# Autodesk Inventor assembly: termoformadora
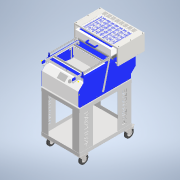
[picture p0: Inventor's stored thumbnail of the model, 180x180]
Saved by Autodesk Inventor 2021 (Build 250183000, 183)
## iProperties
Created: 2021-04-15
Part Number: termoformadora
Document SubType Name: Assembly
Designer: Leonardo Fabio Mercado Benítez
Author: Leonardo Fabio Mercado Benítez
## Documents named in this file (21)
- C:\Users\Nelson\Github\Proyecto_PAI_2021\01 CAD\termoformadora.iam
- C:\Users\Nelson\Github\Proyecto_PAI_2021\01 CAD\soporte_inferior_zona_calor.ipt
- C:\Users\Nelson\Github\Proyecto_PAI_2021\01 CAD\tapa_caja_calor.ipt
- C:\Users\Nelson\Github\Proyecto_PAI_2021\01 CAD\angulo_caja_calor.ipt
- C:\Users\Nelson\Github\Proyecto_PAI_2021\01 CAD\buje_carro_zona_calor.ipt
- C:\Users\Nelson\Github\Proyecto_PAI_2021\01 CAD\barra.ipt
- C:\Users\Nelson\Github\Proyecto_PAI_2021\01 CAD\mango_zona_calor.ipt
- C:\Users\Nelson\Github\Proyecto_PAI_2021\01 CAD\Ensamblaje carcasa control.iam
- C:\Users\Nelson\Github\Proyecto_PAI_2021\01 CAD\soporte_barra.ipt
- C:\Users\Nelson\Github\Proyecto_PAI_2021\01 CAD\ensamble resistencias.iam
- C:\Users\Nelson\Github\Proyecto_PAI_2021\01 CAD\soporte_resistencias.ipt
- C:\Users\Nelson\Github\Proyecto_PAI_2021\01 CAD\Estructura Lámina.iam
- C:\Users\Nelson\Github\Proyecto_PAI_2021\01 CAD\conector_ceramico.ipt
- C:\Users\Nelson\Github\Proyecto_PAI_2021\01 CAD\guarda_conector_ceramico.ipt
- C:\Users\Nelson\Github\Proyecto_PAI_2021\01 CAD\guarda_cables.ipt
- C:\Users\Nelson\Github\Proyecto_PAI_2021\01 CAD\Barras_Soporte_superior.ipt
- C:\Users\Admin\Documents\Inventor\Content Center Files\R2021\es-ES\ISO 7380-1\ISO 7380-1 - M5 x 16.ipt
- C:\Users\Nelson\Github\Proyecto_PAI_2021\01 CAD\DIN EN ISO 7049 - ST2,9 x 6,5 - C - H.ipt
- C:\Users\Nelson\Github\Proyecto_PAI_2021\01 CAD\Tuerca-1_4.ipt
- C:\Users\Nelson\Github\Proyecto_PAI_2021\01 CAD\Tornillo1_4x1_2.ipt
- C:\Users\Nelson\Github\Proyecto_PAI_2021\01 CAD\Ensamblaje_Carcaza_sup_ch.iam
## Components (55 placed, 20 different names)
1. soporte_inferior_zona_calor:1 — Coincidencia:3, Coincidencia:5, Nivelación:3, Nivelación:4, Coincidencia:6, Nivelación:5, Nivelación:6, Coincidencia:15, Insertar:5, Insertar:6, Coincidencia:44, Coincidencia:45, Nivelación:14, Nivelación:15, Ángulo:6, Ángulo:7, Ángulo:8, Ángulo:9, Ángulo:10, Nivelación:16, Coincidencia:56, Nivelación:17
2. tapa_caja_calor:1 — Coincidencia:3, Nivelación:14, Nivelación:15, De rotación:1, De rotación:2, De rotación:3, De rotación:4
3. angulo_caja_calor:1 — Coincidencia:5, Nivelación:3, Nivelación:4, Coincidencia:7, Coincidencia:8, Insertar:1, Insertar:2
4. angulo_caja_calor:2 — Coincidencia:6, Nivelación:5, Nivelación:6, Coincidencia:9, Coincidencia:10, Insertar:3, Insertar:4
5. buje_carro_zona_calor:1 — Coincidencia:9, Insertar:3
6. buje_carro_zona_calor:2 — Coincidencia:8, Insertar:2, Coincidencia:14
7. buje_carro_zona_calor:3 — Coincidencia:10, Insertar:4
8. buje_carro_zona_calor:4 — Coincidencia:7, Insertar:1, Coincidencia:13
9. barra:1 — Coincidencia:13, Coincidencia:21
10. barra:2 — Coincidencia:14, Coincidencia:22
11. mango_zona_calor:1 — Coincidencia:15, Insertar:5, Insertar:6
12. Ensamblaje carcasa control:1 [sub-assembly] — Nivelación:8, Coincidencia:18, Coincidencia:20, Nivelación:9, Coincidencia:23, Coincidencia:33, Nivelación:10, Nivelación:11, Rígido:1, Rígido:2, Rígido:3, Rígido:4
13. soporte_barra:1 — Nivelación:8, Coincidencia:18, Coincidencia:22
14. soporte_barra:2 — Coincidencia:20, Nivelación:9, Coincidencia:21
15. ensamble resistencias:1 [sub-assembly] — Coincidencia:23, Coincidencia:29, Nivelación:12, Nivelación:13, Coincidencia:73, Coincidencia:74, Coincidencia:75, Coincidencia:76, Coincidencia:77, Coincidencia:78, Coincidencia:79, Coincidencia:80, Coincidencia:81, Coincidencia:82, Coincidencia:83, Coincidencia:84
16. soporte_resistencias:1 — Coincidencia:29, Nivelación:12, Nivelación:13, Coincidencia:34, Coincidencia:35, Coincidencia:36, Coincidencia:37, Coincidencia:38, Coincidencia:39, Coincidencia:40, Coincidencia:41, Coincidencia:42, Coincidencia:43, Ángulo:1, Ángulo:2, Ángulo:3, Ángulo:4, Ángulo:5, Coincidencia:44, Coincidencia:45, Coincidencia:61, Coincidencia:62, Coincidencia:63, Coincidencia:64, Coincidencia:65, Coincidencia:66, Coincidencia:67, Coincidencia:68, Coincidencia:69, Coincidencia:70, Coincidencia:71, Coincidencia:72
17. Estructura Lámina:1 [sub-assembly] — Coincidencia:33, Nivelación:10, Nivelación:11
18. conector_ceramico:1 — Coincidencia:37, Coincidencia:42, Ángulo:2, Coincidencia:52, Coincidencia:91
19. conector_ceramico:2 — Coincidencia:36, Coincidencia:41, Ángulo:1, Coincidencia:53, Coincidencia:94
20. conector_ceramico:3 — Coincidencia:34, Coincidencia:39, Ángulo:4, Coincidencia:55, Coincidencia:92
21. conector_ceramico:4 — Coincidencia:38, Coincidencia:43, Ángulo:5, Coincidencia:46, Coincidencia:47, Coincidencia:48, Coincidencia:49, Coincidencia:50, Coincidencia:51, Coincidencia:90
22. conector_ceramico:5 — Coincidencia:35, Coincidencia:40, Ángulo:3, Coincidencia:54, Coincidencia:93
23. guarda_conector_ceramico:1 — Coincidencia:46, Coincidencia:51, Ángulo:10, Coincidencia:89
24. guarda_conector_ceramico:2 — Coincidencia:48, Coincidencia:54, Ángulo:8, Coincidencia:86
25. guarda_conector_ceramico:3 — Coincidencia:47, Coincidencia:52, Ángulo:6, Coincidencia:88
26. guarda_conector_ceramico:4 — Coincidencia:50, Coincidencia:55, Ángulo:9, Coincidencia:87
27. guarda_conector_ceramico:5 — Coincidencia:49, Coincidencia:53, Ángulo:7, Coincidencia:85
28. guarda_cables:1 — Nivelación:16, Coincidencia:56, Nivelación:17
29. Barras_Soporte_superior:1 — Rígido:4
30. Barras_Soporte_superior:2 — Rígido:3
31. Barras_Soporte_superior:3 — Rígido:1
32. Barras_Soporte_superior:4 — Rígido:2, Coincidencia:95
33. ISO 7380-1 M5 x 16:4
34. DIN EN ISO 7049 - C-H ST2,9 x 6,5 - C - H:1 — De rotación:2
35. DIN EN ISO 7049 - C-H ST2,9 x 6,5 - C - H:2 — De rotación:1
36. DIN EN ISO 7049 - C-H ST2,9 x 6,5 - C - H:3 — De rotación:4
37. DIN EN ISO 7049 - C-H ST2,9 x 6,5 - C - H:4 — De rotación:3
38. AS 2465 - Pulgadas 1/4  UNC:1 — Coincidencia:61, Coincidencia:74
39. AS 2465 - Pulgadas 1/4  UNC:2 — Coincidencia:62, Coincidencia:76
40. AS 2465 - Pulgadas 1/4  UNC:3 — Coincidencia:64, Coincidencia:79
41. AS 2465 - Pulgadas 1/4  UNC:4 — Coincidencia:63, Coincidencia:75
42. AS 2465 - Pulgadas 1/4  UNC:5 — Coincidencia:65, Coincidencia:77
43. AS 2465 - Pulgadas 1/4  UNC:6 — Coincidencia:68, Coincidencia:80
44. AS 2465 - Pulgadas 1/4  UNC:7 — Coincidencia:69, Coincidencia:81
45. AS 2465 - Pulgadas 1/4  UNC:8 — Coincidencia:67, Coincidencia:78
46. AS 2465 - Pulgadas 1/4  UNC:9 — Coincidencia:66, Coincidencia:73
47. AS 2465 - Pulgadas 1/4  UNC:10 — Coincidencia:70, Coincidencia:82
48. AS 2465 - Pulgadas 1/4  UNC:11 — Coincidencia:72, Coincidencia:84
49. AS 2465 - Pulgadas 1/4  UNC:12 — Coincidencia:71, Coincidencia:83
50. AS 2465 - Pulgadas 1/4 x 1/2  UNC:1 — Coincidencia:85, Coincidencia:94
51. AS 2465 - Pulgadas 1/4 x 1/2  UNC:2 — Coincidencia:88, Coincidencia:93
52. AS 2465 - Pulgadas 1/4 x 1/2  UNC:3 — Coincidencia:87, Coincidencia:91
53. AS 2465 - Pulgadas 1/4 x 1/2  UNC:4 — Coincidencia:89, Coincidencia:90
54. AS 2465 - Pulgadas 1/4 x 1/2  UNC:5 — Coincidencia:86, Coincidencia:92
55. Ensamblaje_Carcaza_sup_ch:1 [sub-assembly] — Coincidencia:95
## Relationships (113: Mate 75, Flush 14, Angle 10, Insert 6, RevoluteJoint 4, WeldJoint 4)
- Coincidencia:3 [Mate]: soporte_inferior_zona_calor:1 ↔ tapa_caja_calor:1
- Coincidencia:5 [Mate]: soporte_inferior_zona_calor:1 ↔ angulo_caja_calor:1
- Nivelación:3 [Flush]: soporte_inferior_zona_calor:1 ↔ angulo_caja_calor:1
- Nivelación:4 [Flush] (10 mm): soporte_inferior_zona_calor:1 ↔ angulo_caja_calor:1
- Coincidencia:6 [Mate]: soporte_inferior_zona_calor:1 ↔ angulo_caja_calor:2
- Nivelación:5 [Flush]: soporte_inferior_zona_calor:1 ↔ angulo_caja_calor:2
- Nivelación:6 [Flush]: soporte_inferior_zona_calor:1 ↔ angulo_caja_calor:2
- Coincidencia:7 [Mate]: angulo_caja_calor:1 ↔ buje_carro_zona_calor:4
- Coincidencia:8 [Mate]: angulo_caja_calor:1 ↔ buje_carro_zona_calor:2
- Coincidencia:9 [Mate]: angulo_caja_calor:2 ↔ buje_carro_zona_calor:1
- Coincidencia:10 [Mate]: angulo_caja_calor:2 ↔ buje_carro_zona_calor:3
- Insertar:1: angulo_caja_calor:1 ↔ buje_carro_zona_calor:4
- Insertar:2: angulo_caja_calor:1 ↔ buje_carro_zona_calor:2
- Insertar:3: angulo_caja_calor:2 ↔ buje_carro_zona_calor:1
- Insertar:4: angulo_caja_calor:2 ↔ buje_carro_zona_calor:3
- Coincidencia:13 [Mate]: buje_carro_zona_calor:4 ↔ barra:1
- Coincidencia:14 [Mate]: buje_carro_zona_calor:2 ↔ barra:2
- Coincidencia:15 [Mate]: soporte_inferior_zona_calor:1 ↔ mango_zona_calor:1
- Insertar:5: soporte_inferior_zona_calor:1 ↔ mango_zona_calor:1
- Insertar:6: soporte_inferior_zona_calor:1 ↔ mango_zona_calor:1
- Nivelación:8 [Flush] (5 mm): Ensamblaje carcasa control:1 ↔ soporte_barra:1
- Coincidencia:18 [Mate]: Ensamblaje carcasa control:1 ↔ soporte_barra:1
- Coincidencia:20 [Mate]: Ensamblaje carcasa control:1 ↔ soporte_barra:2
- Nivelación:9 [Flush] (5 mm): Ensamblaje carcasa control:1 ↔ soporte_barra:2
- Coincidencia:21 [Mate]: barra:1 ↔ soporte_barra:2
- Coincidencia:22 [Mate]: barra:2 ↔ soporte_barra:1
- Coincidencia:23 [Mate] (106 mm): Ensamblaje carcasa control:1 ↔ ensamble resistencias:1
- Coincidencia:29 [Mate]: ensamble resistencias:1 ↔ soporte_resistencias:1
- Coincidencia:33 [Mate]: Ensamblaje carcasa control:1 ↔ Estructura Lámina:1
- Nivelación:10 [Flush] (10 mm): Ensamblaje carcasa control:1 ↔ Estructura Lámina:1
- Nivelación:11 [Flush]: Ensamblaje carcasa control:1 ↔ Estructura Lámina:1
- Nivelación:12 [Flush] (33.5 mm): ensamble resistencias:1 ↔ soporte_resistencias:1
- Nivelación:13 [Flush] (34 mm): ensamble resistencias:1 ↔ soporte_resistencias:1
- Coincidencia:34 [Mate]: soporte_resistencias:1 ↔ conector_ceramico:3
- Coincidencia:35 [Mate]: soporte_resistencias:1 ↔ conector_ceramico:5
- Coincidencia:36 [Mate]: soporte_resistencias:1 ↔ conector_ceramico:2
- Coincidencia:37 [Mate]: soporte_resistencias:1 ↔ conector_ceramico:1
- Coincidencia:38 [Mate]: soporte_resistencias:1 ↔ conector_ceramico:4
- Coincidencia:39 [Mate]: soporte_resistencias:1 ↔ conector_ceramico:3
- Coincidencia:40 [Mate]: soporte_resistencias:1 ↔ conector_ceramico:5
- Coincidencia:41 [Mate]: soporte_resistencias:1 ↔ conector_ceramico:2
- Coincidencia:42 [Mate]: soporte_resistencias:1 ↔ conector_ceramico:1
- Coincidencia:43 [Mate]: soporte_resistencias:1 ↔ conector_ceramico:4
- Ángulo:1 [Angle] (0 deg): soporte_resistencias:1 ↔ conector_ceramico:2
- Ángulo:2 [Angle] (0 deg): soporte_resistencias:1 ↔ conector_ceramico:1
- Ángulo:3 [Angle] (0 deg): soporte_resistencias:1 ↔ conector_ceramico:5
- Ángulo:4 [Angle] (0 deg): soporte_resistencias:1 ↔ conector_ceramico:3
- Ángulo:5 [Angle] (0 deg): soporte_resistencias:1 ↔ conector_ceramico:4
- Coincidencia:44 [Mate] (0.5 mm): soporte_inferior_zona_calor:1 ↔ soporte_resistencias:1
- Coincidencia:45 [Mate] (0.5 mm): soporte_inferior_zona_calor:1 ↔ soporte_resistencias:1
- Nivelación:14 [Flush] (25.4 mm): soporte_inferior_zona_calor:1 ↔ tapa_caja_calor:1
- Nivelación:15 [Flush] (31.75 mm): soporte_inferior_zona_calor:1 ↔ tapa_caja_calor:1
- Coincidencia:46 [Mate]: conector_ceramico:4 ↔ guarda_conector_ceramico:1
- Coincidencia:47 [Mate]: conector_ceramico:4 ↔ guarda_conector_ceramico:3
- Coincidencia:48 [Mate]: conector_ceramico:4 ↔ guarda_conector_ceramico:2
- Coincidencia:49 [Mate]: conector_ceramico:4 ↔ guarda_conector_ceramico:5
- Coincidencia:50 [Mate]: conector_ceramico:4 ↔ guarda_conector_ceramico:4
- Coincidencia:51 [Mate]: conector_ceramico:4 ↔ guarda_conector_ceramico:1
- Coincidencia:52 [Mate]: conector_ceramico:1 ↔ guarda_conector_ceramico:3
- Coincidencia:53 [Mate]: conector_ceramico:2 ↔ guarda_conector_ceramico:5
- Coincidencia:54 [Mate]: conector_ceramico:5 ↔ guarda_conector_ceramico:2
- Coincidencia:55 [Mate]: conector_ceramico:3 ↔ guarda_conector_ceramico:4
- Ángulo:6 [Angle] (0 deg): soporte_inferior_zona_calor:1 ↔ guarda_conector_ceramico:3
- Ángulo:7 [Angle] (0 deg): soporte_inferior_zona_calor:1 ↔ guarda_conector_ceramico:5
- Ángulo:8 [Angle] (0 deg): soporte_inferior_zona_calor:1 ↔ guarda_conector_ceramico:2
- Ángulo:9 [Angle] (0 deg): soporte_inferior_zona_calor:1 ↔ guarda_conector_ceramico:4
- Ángulo:10 [Angle] (0 deg): soporte_inferior_zona_calor:1 ↔ guarda_conector_ceramico:1
- Nivelación:16 [Flush]: soporte_inferior_zona_calor:1 ↔ guarda_cables:1
- Coincidencia:56 [Mate]: soporte_inferior_zona_calor:1 ↔ guarda_cables:1
- Nivelación:17 [Flush]: soporte_inferior_zona_calor:1 ↔ guarda_cables:1
- De rotación:1 [RevoluteJoint]: tapa_caja_calor:1 ↔ DIN EN ISO 7049 - C-H ST2,9 x 6,5 - C - H:2
- De rotación:2 [RevoluteJoint]: tapa_caja_calor:1 ↔ DIN EN ISO 7049 - C-H ST2,9 x 6,5 - C - H:1
- De rotación:3 [RevoluteJoint]: tapa_caja_calor:1 ↔ DIN EN ISO 7049 - C-H ST2,9 x 6,5 - C - H:4
- De rotación:4 [RevoluteJoint]: tapa_caja_calor:1 ↔ DIN EN ISO 7049 - C-H ST2,9 x 6,5 - C - H:3
- Coincidencia:61 [Mate]: soporte_resistencias:1 ↔ AS 2465 - Pulgadas 1/4  UNC:1
- Coincidencia:62 [Mate]: soporte_resistencias:1 ↔ AS 2465 - Pulgadas 1/4  UNC:2
- Coincidencia:63 [Mate]: soporte_resistencias:1 ↔ AS 2465 - Pulgadas 1/4  UNC:4
- Coincidencia:64 [Mate]: soporte_resistencias:1 ↔ AS 2465 - Pulgadas 1/4  UNC:3
- Coincidencia:65 [Mate]: soporte_resistencias:1 ↔ AS 2465 - Pulgadas 1/4  UNC:5
- Coincidencia:66 [Mate]: soporte_resistencias:1 ↔ AS 2465 - Pulgadas 1/4  UNC:9
- Coincidencia:67 [Mate]: soporte_resistencias:1 ↔ AS 2465 - Pulgadas 1/4  UNC:8
- Coincidencia:68 [Mate]: soporte_resistencias:1 ↔ AS 2465 - Pulgadas 1/4  UNC:6
- Coincidencia:69 [Mate]: soporte_resistencias:1 ↔ AS 2465 - Pulgadas 1/4  UNC:7
- Coincidencia:70 [Mate]: soporte_resistencias:1 ↔ AS 2465 - Pulgadas 1/4  UNC:10
- Coincidencia:71 [Mate]: soporte_resistencias:1 ↔ AS 2465 - Pulgadas 1/4  UNC:12
- Coincidencia:72 [Mate]: soporte_resistencias:1 ↔ AS 2465 - Pulgadas 1/4  UNC:11
- Coincidencia:73 [Mate]: ensamble resistencias:1 ↔ AS 2465 - Pulgadas 1/4  UNC:9
- Coincidencia:74 [Mate]: ensamble resistencias:1 ↔ AS 2465 - Pulgadas 1/4  UNC:1
- Coincidencia:75 [Mate]: ensamble resistencias:1 ↔ AS 2465 - Pulgadas 1/4  UNC:4
- Coincidencia:76 [Mate]: ensamble resistencias:1 ↔ AS 2465 - Pulgadas 1/4  UNC:2
- Coincidencia:77 [Mate]: ensamble resistencias:1 ↔ AS 2465 - Pulgadas 1/4  UNC:5
- Coincidencia:78 [Mate]: ensamble resistencias:1 ↔ AS 2465 - Pulgadas 1/4  UNC:8
- Coincidencia:79 [Mate]: ensamble resistencias:1 ↔ AS 2465 - Pulgadas 1/4  UNC:3
- Coincidencia:80 [Mate]: ensamble resistencias:1 ↔ AS 2465 - Pulgadas 1/4  UNC:6
- Coincidencia:81 [Mate]: ensamble resistencias:1 ↔ AS 2465 - Pulgadas 1/4  UNC:7
- Coincidencia:82 [Mate]: ensamble resistencias:1 ↔ AS 2465 - Pulgadas 1/4  UNC:10
- Coincidencia:83 [Mate]: ensamble resistencias:1 ↔ AS 2465 - Pulgadas 1/4  UNC:12
- Coincidencia:84 [Mate]: ensamble resistencias:1 ↔ AS 2465 - Pulgadas 1/4  UNC:11
- Coincidencia:85 [Mate]: guarda_conector_ceramico:5 ↔ AS 2465 - Pulgadas 1/4 x 1/2  UNC:1
- Coincidencia:86 [Mate]: guarda_conector_ceramico:2 ↔ AS 2465 - Pulgadas 1/4 x 1/2  UNC:5
- Coincidencia:87 [Mate]: guarda_conector_ceramico:4 ↔ AS 2465 - Pulgadas 1/4 x 1/2  UNC:3
- Coincidencia:88 [Mate]: guarda_conector_ceramico:3 ↔ AS 2465 - Pulgadas 1/4 x 1/2  UNC:2
- Coincidencia:89 [Mate]: guarda_conector_ceramico:1 ↔ AS 2465 - Pulgadas 1/4 x 1/2  UNC:4
- Coincidencia:90 [Mate]: conector_ceramico:4 ↔ AS 2465 - Pulgadas 1/4 x 1/2  UNC:4
- Coincidencia:91 [Mate]: conector_ceramico:1 ↔ AS 2465 - Pulgadas 1/4 x 1/2  UNC:3
- Coincidencia:92 [Mate]: conector_ceramico:3 ↔ AS 2465 - Pulgadas 1/4 x 1/2  UNC:5
- Coincidencia:93 [Mate]: conector_ceramico:5 ↔ AS 2465 - Pulgadas 1/4 x 1/2  UNC:2
- Coincidencia:94 [Mate]: conector_ceramico:2 ↔ AS 2465 - Pulgadas 1/4 x 1/2  UNC:1
- Rígido:1 [WeldJoint]: Ensamblaje carcasa control:1 ↔ Barras_Soporte_superior:3
- Rígido:2 [WeldJoint]: Ensamblaje carcasa control:1 ↔ Barras_Soporte_superior:4
- Rígido:3 [WeldJoint]: Ensamblaje carcasa control:1 ↔ Barras_Soporte_superior:2
- Rígido:4 [WeldJoint]: Ensamblaje carcasa control:1 ↔ Barras_Soporte_superior:1
- Coincidencia:95 [Mate]: Barras_Soporte_superior:4 ↔ Ensamblaje_Carcaza_sup_ch:1
